# Autodesk Inventor assembly: 部件2
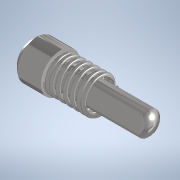
[picture p0: Inventor's stored thumbnail of the model, 180x180]
Saved by Autodesk Inventor 2022 (Build 260153000, 153)
## iProperties
Created: 2023-01-11
Part Number: 部件2
Document SubType Name: Assembly
Designer: Lzy18
Author: Lzy18
## Documents named in this file (3)
- C:\Users\Lzy18\Desktop\夹体\部件2.iam
- C:\Users\Lzy18\Desktop\夹体\7-顶轴.ipt
- C:\Users\Lzy18\Desktop\夹体\Compress Spring12.ipt
## Components (2 placed, 2 different names)
1. 7-顶轴:1 — 表面齐平:1
2. Compress Spring1:1 — 配合:1, 表面齐平:1
## Relationships (2: Mate 1, Flush 1)
- 配合:1 [Mate]: Compress Spring1:1
- 表面齐平:1 [Flush]: 7-顶轴:1 ↔ Compress Spring1:1
